# Autodesk Inventor assembly: cam-flying
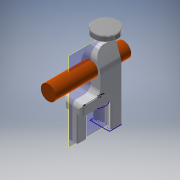
[picture p0: Inventor's stored thumbnail of the model, 180x180]
Saved by Autodesk Inventor 2016 (Build 200138000, 138)
## iProperties
Created: 2015-05-15
Part Number: cam-flying
Document SubType Name: Assembly
Designer: as
Author: as
## Documents named in this file (4)
- C:\Users\as\Documents\Inventor\mintplacer-export\render\cam-flying.iam
- C:\Users\as\Documents\Inventor\mintplacer-export\render\cam-flying-mount.ipt
- C:\Users\as\Documents\Inventor\mintplacer-export\render\flying-cam-10mm.ipt
- C:\Users\as\Documents\Inventor\Content Center Files\R2016\en-US\DIN 653\DIN 653 - M4 x 10.ipt
## Components (3 placed, 3 different names)
1. cam-flying-mount:1 — Mate:1, Insert:1, Mate:2, Angle:1, Flush:1
2. flying-cam-10mm:1 — Mate:1, Flush:1
3. DIN 653 M4 x 10:1 — Insert:1
## Relationships (5: Mate 2, Insert 1, Angle 1, Flush 1)
- Mate:1: cam-flying-mount:1 ↔ flying-cam-10mm:1
- Insert:1 (-6 mm): cam-flying-mount:1 ↔ DIN 653 M4 x 10:1
- Mate:2: cam-flying-mount:1
- Angle:1 (0 deg): cam-flying-mount:1
- Flush:1 (-8 mm): cam-flying-mount:1 ↔ flying-cam-10mm:1
